# Autodesk Inventor assembly: FullLegAssembly
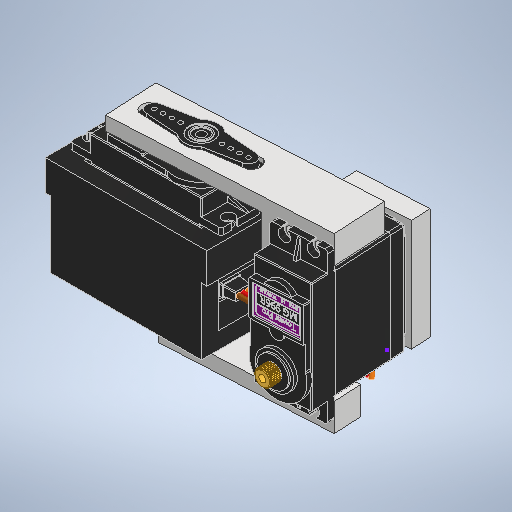
[picture p0: Inventor's stored thumbnail of the model, 512x512]
Saved by Autodesk Inventor 2025 (Build 290162000, 162)
## iProperties
Created: 2024-09-10
Part Number: FullLegAssembly
Document SubType Name: Assembly
Designer: omiye
Author: omiye
## Documents named in this file (5)
- C:\Users\7008661\Downloads\hexapod\legModels\FullLegAssembly.iam
- C:\Users\7008661\Downloads\hexapod\legModels\MG996RServo.ipt
- C:\Users\7008661\Downloads\hexapod\legModels\MG996RServoHolder.ipt
- C:\Users\7008661\Downloads\hexapod\legModels\straightServoHorn.ipt
- C:\Users\7008661\Downloads\hexapod\legModels\miscStuff\coxaModel.ipt
## Components (5 placed, 4 different names)
1. MG996RServo:1 — Mate:1, Mate:2, Mate:5, Mate:6, Mate:9, Mate:10, Mate:11, Mate:12
2. MG996RServoHolder:1 — Mate:1, Mate:2, Mate:9, Mate:10, Mate:11, Mate:12
3. straightServoHorn:1 — Mate:5, Mate:6, Mate:13, Mate:14, Mate:15, Mate:16
4. coxaModel:1 — Mate:13, Mate:14, Mate:15, Mate:16, Mate:17, Mate:18, Mate:19, Mate:20
5. MG996RServo:2 — Mate:17, Mate:18, Mate:19, Mate:20
## Relationships (16: Mate 16)
- Mate:1: MG996RServo:1 ↔ MG996RServoHolder:1
- Mate:2: MG996RServo:1 ↔ MG996RServoHolder:1
- Mate:5: MG996RServo:1 ↔ straightServoHorn:1
- Mate:6: MG996RServo:1 ↔ straightServoHorn:1
- Mate:9: MG996RServo:1 ↔ MG996RServoHolder:1
- Mate:10: MG996RServo:1 ↔ MG996RServoHolder:1
- Mate:11: MG996RServo:1 ↔ MG996RServoHolder:1
- Mate:12: MG996RServo:1 ↔ MG996RServoHolder:1
- Mate:13: straightServoHorn:1 ↔ coxaModel:1
- Mate:14: straightServoHorn:1 ↔ coxaModel:1
- Mate:15: straightServoHorn:1 ↔ coxaModel:1
- Mate:16: straightServoHorn:1 ↔ coxaModel:1
- Mate:17: coxaModel:1 ↔ MG996RServo:2
- Mate:18: coxaModel:1 ↔ MG996RServo:2
- Mate:19: coxaModel:1 ↔ MG996RServo:2
- Mate:20: coxaModel:1 ↔ MG996RServo:2
